# Autodesk Inventor assembly: 无碳小车装配体
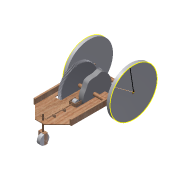
[picture p0: Inventor's stored thumbnail of the model, 180x180]
Saved by Autodesk Inventor 2013 (Build 170138000, 138)
## iProperties
Created: 2012-10-03
Part Number: 无碳小车装配体
Document SubType Name: Assembly
Designer: Zhensheng
Mass: 1427.51 g
Surface Area: 1958.94 cm^2
Volume: 619.252 cm^3
Density: 2.30522 g/cm^3
Author: Zhensheng
## Documents named in this file (17)
- E:\inventor\无碳小车\无碳小车装配体.iam
- E:\inventor\无碳小车\底板.ipt
- E:\inventor\无碳小车\主轴.ipt
- E:\inventor\无碳小车\带轮.ipt
- E:\inventor\无碳小车\后轮.ipt
- E:\inventor\无碳小车\副轴.ipt
- E:\inventor\无碳小车\齿轮套筒.ipt
- E:\inventor\无碳小车\无碳小车装配体\设计加速器\正齿轮1.iam
- E:\inventor\无碳小车\凸轮套筒.ipt
- E:\inventor\无碳小车\凸轮.ipt
- E:\inventor\无碳小车\顶杆.ipt
- E:\inventor\无碳小车\滚子.ipt
- E:\inventor\无碳小车\连接销4.ipt
- E:\inventor\无碳小车\顶杆支架.ipt
- E:\inventor\无碳小车\曲柄-新.ipt
- E:\inventor\无碳小车\前轮.ipt
- E:\inventor\无碳小车\前轮撑杆.ipt
## Components (19 placed, 16 different names)
1. 底板:1 — 轴-后轮, 后轮对称, 带轮中, 表面齐平:4, 配合:6, 配合:8, 配合:10, 配合:15, 顶杆中, 支架中, 配合:23, 配合:24, 前轮, 配合:33
2. 主轴:1 — 轴-后轮, 后轮对称, 表面齐平:2, 配合:2, 表面齐平:3, 配合:3, 配合:4, 配合:7, 配合:11
3. 带轮:1 — 配合:4, 带轮中
4. 后轮:1 — 表面齐平:2, 配合:2
5. 后轮:2 — 表面齐平:3, 配合:3
6. 副轴:1 — 表面齐平:4, 配合:6, 配合:9, 配合:13, 配合:16, 配合:18
7. 齿轮套筒:1 — 配合:7, 配合:8, 配合:12
8. 齿轮套筒:2 — 配合:9, 配合:10, 配合:14
9. 正齿轮:1 [sub-assembly] — 配合:11, 配合:12, 配合:13, 配合:14
10. 凸轮套筒:1 — 配合:15, 配合:16, 配合:17
11. 凸轮:2 — 配合:17, 配合:18
12. 顶杆:1 — 表面齐平:5, 配合:19, 滚子中, 配合:26, 配合:27, 曲柄中
13. 滚子:1 — 滚子中, 配合:21, 顶杆中
14. 连接销4:1 — 表面齐平:5, 配合:19, 配合:21
15. 顶杆支架:1 — 配合:23, 表面齐平:6, 支架中, 配合:26
16. 顶杆支架:2 — 配合:24, 表面齐平:6
17. 曲柄-新:1 — 配合:27, 曲柄中, 配合:31
18. 前轮:1 — 配合:29, 前轮中, 前轮
19. 前轮撑杆:1 — 配合:29, 前轮中, 配合:31, 配合:33
## Relationships (39: Mate 33, Flush 6)
- 轴-后轮 [Mate]: 底板:1 ↔ 主轴:1
- 后轮对称 [Flush] (-15 mm): 底板:1 ↔ 主轴:1
- 滚子中 [Mate] (4 mm): 顶杆:1 ↔ 滚子:1
- 表面齐平:2 [Flush]: 主轴:1 ↔ 后轮:1
- 带轮中 [Mate] (5 mm): 底板:1 ↔ 带轮:1
- 顶杆中 [Mate] (40 mm): 底板:1 ↔ 滚子:1
- 支架中 [Mate] (41 mm): 底板:1 ↔ 顶杆支架:1
- 曲柄中 [Mate] (0.5 mm): 顶杆:1 ↔ 曲柄-新:1
- 前轮中 [Mate] (4 mm): 前轮:1 ↔ 前轮撑杆:1
- 前轮 [Mate] (50 mm): 底板:1 ↔ 前轮:1
- 配合:2 [Mate]: 主轴:1 ↔ 后轮:1
- 表面齐平:3 [Flush]: 主轴:1 ↔ 后轮:2
- 配合:3 [Mate]: 主轴:1 ↔ 后轮:2
- 配合:4 [Mate]: 主轴:1 ↔ 带轮:1
- 表面齐平:4 [Flush]: 底板:1 ↔ 副轴:1
- 配合:6 [Mate]: 底板:1 ↔ 副轴:1
- 配合:7 [Mate]: 主轴:1 ↔ 齿轮套筒:1
- 配合:8 [Mate]: 底板:1 ↔ 齿轮套筒:1
- 配合:9 [Mate]: 副轴:1 ↔ 齿轮套筒:2
- 配合:10 [Mate]: 底板:1 ↔ 齿轮套筒:2
- 配合:11 [Mate]: 主轴:1 ↔ 正齿轮:1
- 配合:12 [Mate]: 齿轮套筒:1 ↔ 正齿轮:1
- 配合:13 [Mate]: 副轴:1 ↔ 正齿轮:1
- 配合:14 [Mate]: 齿轮套筒:2 ↔ 正齿轮:1
- 配合:15 [Mate]: 底板:1 ↔ 凸轮套筒:1
- 配合:16 [Mate]: 副轴:1 ↔ 凸轮套筒:1
- 配合:17 [Mate]: 凸轮套筒:1 ↔ 凸轮:2
- 配合:18 [Mate]: 副轴:1 ↔ 凸轮:2
- 表面齐平:5 [Flush]: 顶杆:1 ↔ 连接销4:1
- 配合:19 [Mate]: 顶杆:1 ↔ 连接销4:1
- 配合:21 [Mate]: 滚子:1 ↔ 连接销4:1
- 配合:23 [Mate]: 底板:1 ↔ 顶杆支架:1
- 配合:24 [Mate]: 底板:1 ↔ 顶杆支架:2
- 表面齐平:6 [Flush]: 顶杆支架:1 ↔ 顶杆支架:2
- 配合:26 [Mate]: 顶杆:1 ↔ 顶杆支架:1
- 配合:27 [Mate]: 顶杆:1 ↔ 曲柄-新:1
- 配合:29 [Mate]: 前轮:1 ↔ 前轮撑杆:1
- 配合:31 [Mate]: 曲柄-新:1 ↔ 前轮撑杆:1
- 配合:33 [Mate]: 底板:1 ↔ 前轮撑杆:1
## Named parameters: 顶杆中 = 40 mm, 曲柄杆 = 0.5 mm
